# Autodesk Inventor assembly: CIMpleBoxStandalone
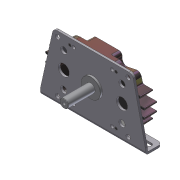
[picture p0: Inventor's stored thumbnail of the model, 180x180]
Saved by Autodesk Inventor 2012 (Build 160160000, 160)
## iProperties
Created: 2012-02-26
Part Number: CIMpleBoxStandalone
Document SubType Name: Assembly
Designer: JesseK
Author: JesseK
## Documents named in this file (5)
- Z:\UserData\Documents\Inventor\team1885frc\AndyMark\CIMpleBox\CIMpleBoxStandalone.iam
- Z:\UserData\Documents\Inventor\team1885frc\AndyMark\CIMpleBox\Single_d02.ipt
- Z:\UserData\Documents\Inventor\team1885frc\AndyMark\CIMpleBox\Single_d01.ipt
- Z:\UserData\Documents\Inventor\team1885frc\AndyMark\CIMpleBox\fr-8-zz.ipt
- Z:\UserData\Documents\Inventor\team1885frc\AndyMark\CIMpleBox\Single_d03.ipt
## Components (4 placed, 4 different names)
1. Single_d02:1 — Mate:1, Mate:2, Mate:3, Mate:4, Mate:5
2. Single_d01:1 — Mate:1, Mate:2, Mate:3
3. fr-8-zz:1 — Mate:4, Mate:5, Mate:6, Mate:7
4. Single_d03:1 — Mate:6, Mate:7
## Relationships (7: Mate 7)
- Mate:1: Single_d02:1 ↔ Single_d01:1
- Mate:2: Single_d02:1 ↔ Single_d01:1
- Mate:3: Single_d02:1 ↔ Single_d01:1
- Mate:4: Single_d02:1 ↔ fr-8-zz:1
- Mate:5: Single_d02:1 ↔ fr-8-zz:1
- Mate:6: fr-8-zz:1 ↔ Single_d03:1
- Mate:7: fr-8-zz:1 ↔ Single_d03:1
